# Autodesk Inventor assembly: Tolva
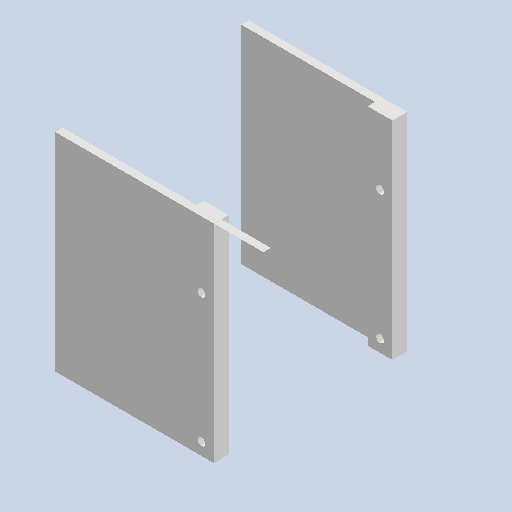
[picture p0: Inventor's stored thumbnail of the model, 512x512]
Saved by Autodesk Inventor 2024 (Build 280153000, 153)
## iProperties
Created: 2025-03-02
Part Number: Tolva
Document SubType Name: Assembly
Designer: sergi
Author: sergi
## Documents named in this file (3)
- C:\Users\sergi\OneDrive\Escritorio\GitHub\16. Catapult\Inventor\Tolva.iam
- C:\Users\sergi\OneDrive\Escritorio\GitHub\16. Catapult\Inventor\Lateral izquierdo.ipt
- C:\Users\sergi\OneDrive\Escritorio\GitHub\16. Catapult\Inventor\Lateral derecho.ipt
## Components (2 placed, 2 different names)
1. Lateral izquierdo:1 — Coincidencia:1, Nivelación:1, Nivelación:2
2. Lateral derecho:1 — Coincidencia:1, Nivelación:1, Nivelación:2
## Relationships (3: Flush 2, Mate 1)
- Coincidencia:1 [Mate] (72 mm): Lateral izquierdo:1 ↔ Lateral derecho:1
- Nivelación:1 [Flush]: Lateral izquierdo:1 ↔ Lateral derecho:1
- Nivelación:2 [Flush]: Lateral izquierdo:1 ↔ Lateral derecho:1
